# Autodesk Inventor assembly: CycloidalDrive2
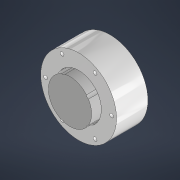
[picture p0: Inventor's stored thumbnail of the model, 180x180]
Saved by Autodesk Inventor 2021 (Build 250183000, 183)
## iProperties
Created: 2022-10-07
Part Number: CycloidalDrive2
Document SubType Name: Assembly
Designer: MicnedSQ
Author: MicnedSQ
## Documents named in this file (3)
- C:\Users\MicnedSQ\Desktop\RobotArmV1\RotatingBase\CycloidalDrive\CycloidalDrive2.iam
- C:\Users\MicnedSQ\Desktop\RobotArmV1\RotatingBase\CycloidalDrive\Bottom.ipt
- C:\Users\MicnedSQ\Desktop\RobotArmV1\RotatingBase\CycloidalDrive\OutputShaft.iam
## Components (2 placed, 2 different names)
1. Bottom:1 — Obrotowe:1
2. OutputShaft:1 [sub-assembly] — Obrotowe:1
## Relationships (1: RevoluteJoint 1)
- Obrotowe:1 [RevoluteJoint]: Bottom:1 ↔ OutputShaft:1
